# Autodesk Inventor assembly: robotface
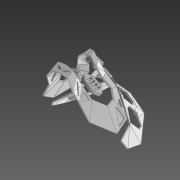
[picture p0: Inventor's stored thumbnail of the model, 180x180]
Saved by Autodesk Inventor 2020 (Build 240168000, 168)
## iProperties
Created: 2021-06-30
Part Number: robotface
Document SubType Name: Assembly
Designer: valer
Author: valer
## Documents named in this file (5)
- C:\Users\valer\Desktop\drummingrobot\design\robotface\robotface.iam
- C:\Users\valer\Desktop\drummingrobot\design\robotface\robotface-final.ipt
- C:\Users\valer\Desktop\drummingrobot\src\parts\external\HingedThreadedStandoffPart2.ipt
- C:\Users\valer\Desktop\drummingrobot\src\parts\external\HingedThreadedStandoffPart1.ipt
- C:\Users\valer\Desktop\drummingrobot\design\robotface\TongueMount.ipt
## Components (8 placed, 4 different names)
1. robotface-final:1 — Mate:7, Mate:8, Mate:9, Mate:10, Mate:11, Mate:12, Angle:3, Angle:4
2. HingedThreadedStandoffPart2:1 — Mate:1, Mate:2, Angle:1, Angle:2, Mate:15, Mate:16
3. HingedThreadedStandoffPart1:1 — Mate:1, Mate:2, Mate:7, Mate:8, Angle:4
4. HingedThreadedStandoffPart2:2 — Mate:3, Mate:4, Mate:9, Mate:10
5. HingedThreadedStandoffPart1:2 — Mate:3, Mate:4, Angle:1, Mate:17
6. HingedThreadedStandoffPart2:3 — Mate:5, Mate:6, Mate:11, Mate:12, Angle:3
7. HingedThreadedStandoffPart1:3 — Mate:5, Mate:6, Angle:2
8. TongueMount:1 — Mate:15, Mate:16, Mate:17
## Relationships (19: Mate 15, Angle 4)
- Mate:1: HingedThreadedStandoffPart2:1 ↔ HingedThreadedStandoffPart1:1
- Mate:2: HingedThreadedStandoffPart2:1 ↔ HingedThreadedStandoffPart1:1
- Mate:3: HingedThreadedStandoffPart2:2 ↔ HingedThreadedStandoffPart1:2
- Mate:4: HingedThreadedStandoffPart2:2 ↔ HingedThreadedStandoffPart1:2
- Mate:5: HingedThreadedStandoffPart2:3 ↔ HingedThreadedStandoffPart1:3
- Mate:6: HingedThreadedStandoffPart2:3 ↔ HingedThreadedStandoffPart1:3
- Mate:7: robotface-final:1 ↔ HingedThreadedStandoffPart1:1
- Mate:8: robotface-final:1 ↔ HingedThreadedStandoffPart1:1
- Mate:9: robotface-final:1 ↔ HingedThreadedStandoffPart2:2
- Mate:10: robotface-final:1 ↔ HingedThreadedStandoffPart2:2
- Mate:11: robotface-final:1 ↔ HingedThreadedStandoffPart2:3
- Mate:12: robotface-final:1 ↔ HingedThreadedStandoffPart2:3
- Angle:1 (0 deg): HingedThreadedStandoffPart2:1 ↔ HingedThreadedStandoffPart1:2
- Angle:2 (0 deg): HingedThreadedStandoffPart2:1 ↔ HingedThreadedStandoffPart1:3
- Angle:3 (0 deg): robotface-final:1 ↔ HingedThreadedStandoffPart2:3
- Angle:4 (0 deg): robotface-final:1 ↔ HingedThreadedStandoffPart1:1
- Mate:15: HingedThreadedStandoffPart2:1 ↔ TongueMount:1
- Mate:16: HingedThreadedStandoffPart2:1 ↔ TongueMount:1
- Mate:17: HingedThreadedStandoffPart1:2 ↔ TongueMount:1
